# Autodesk Inventor assembly: Body
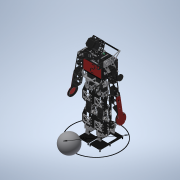
[picture p0: Inventor's stored thumbnail of the model, 180x180]
Saved by Autodesk Inventor 2020.4 (Build 244396000, 396)
## iProperties
Created: 2021-09-30
Part Number: Body
Document SubType Name: Assembly
Designer: Masato Kubotera
Mass: 3701.21 g
Surface Area: 13379.4 cm^2
Volume: 3277.75 cm^3
Density: 1.12919 g/cm^3
Author: Masato Kubotera
## Documents named in this file (5)
- C:\Users\Masato\Documents\Inventor\CIT Brains_Inventor\SUSTAINA-OP\Body.iam
- C:\Users\Masato\Documents\Inventor\CIT Brains_Inventor\SUSTAINA-OP\UpperBody\UpperBody.iam
- C:\Users\Masato\Documents\Inventor\CIT Brains_Inventor\SUSTAINA-OP\LowerBody\LowerBody.iam
- C:\Users\Masato\Documents\Inventor\CIT Brains_Inventor\SUSTAINA-OP\ReadyMade\Ball.ipt
- C:\Users\Masato\Documents\Inventor\CIT Brains_Inventor\SUSTAINA-OP\RegulationCylinder.ipt
## Components (5 placed, 4 different names)
1. UpperBody:1 [sub-assembly] — 挿入:1, フラッシュ:1, 挿入:2
2. LowerBody:1 [sub-assembly] — 挿入:1, フラッシュ:3, メイト:3, 角度:1
3. LowerBody:2 [sub-assembly] — 挿入:2, 角度:1
4. Ball:1 — 正接:1, メイト:1, メイト:2
5. RegulationCylinder:1 — メイト:4, メイト:5
## Relationships (11: Mate 5, Insert 2, Flush 2, Tangent 1, Angle 1)
- 正接:1 [Tangent]: Ball:1
- メイト:1 [Mate] (200 mm): Ball:1
- メイト:2 [Mate]: Ball:1
- 挿入:1 [Insert]: UpperBody:1 ↔ LowerBody:1
- フラッシュ:1 [Flush]: UpperBody:1
- フラッシュ:3 [Flush]: LowerBody:1
- メイト:3 [Mate]: LowerBody:1
- 挿入:2 [Insert]: UpperBody:1 ↔ LowerBody:2
- 角度:1 [Angle] (0 deg): LowerBody:1 ↔ LowerBody:2
- メイト:4 [Mate]: RegulationCylinder:1
- メイト:5 [Mate]: RegulationCylinder:1
